# Autodesk Inventor assembly: body
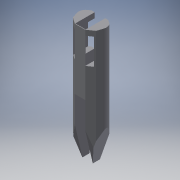
[picture p0: Inventor's stored thumbnail of the model, 180x180]
Saved by Autodesk Inventor 2016 (Build 200138000, 138)
## iProperties
Created: 2019-01-22
Part Number: body
Document SubType Name: Assembly
Designer: LinJie
Author: LinJie
## Documents named in this file (4)
- C:\Users\LinJie\Documents\Inventor\EA Water project\body.iam
- C:\Users\LinJie\Documents\Inventor\EA Water project\bodybase.ipt
- C:\Users\LinJie\Documents\Inventor\EA Water project\bodyside.ipt
- C:\Users\LinJie\Documents\Inventor\EA Water project\bodyside_MIR2.ipt
## Components (3 placed, 3 different names)
1. bodybase:1 — Mate:1, Flush:1, Angle:1
2. bodyside:1 — Mate:1, Flush:1, Angle:1
3. bodyside_MIR2:1
## Relationships (3: Mate 1, Flush 1, Angle 1)
- Mate:1: bodybase:1 ↔ bodyside:1
- Flush:1: bodybase:1 ↔ bodyside:1
- Angle:1 (90 deg): bodybase:1 ↔ bodyside:1
